# Autodesk Inventor assembly: rcache
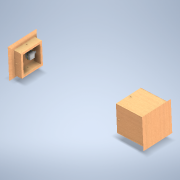
[picture p0: Inventor's stored thumbnail of the model, 180x180]
Saved by Autodesk Inventor 2021 (Build 250183000, 183)
## iProperties
Created: 2020-06-13
Part Number: rcache
Document SubType Name: Assembly
Designer: Yatekii
Author: Yatekii
## Documents named in this file (5)
- C:\Users\Yatekii\repos\rcache\cad\rcache.iam
- C:\Users\Yatekii\repos\rcache\cad\inner.iam
- C:\Users\Yatekii\repos\rcache\cad\outer.iam
- C:\Users\Yatekii\repos\rcache\cad\solenoid\solenoid.iam
- C:\Users\Yatekii\repos\rcache\cad\locker.ipt
## Components (4 placed, 4 different names)
1. inner:1 [sub-assembly] — Slider:1
2. outer:1 [sub-assembly] — Mate:2, Slider:1, Mate:3, Mate:4
3. solenoid:1 [sub-assembly] — Rigid:1, Mate:3, Mate:4
4. locker:1 — Rigid:1, Mate:2
## Relationships (5: Mate 3, WeldJoint 1, TranslationJoint 1)
- Rigid:1 [WeldJoint]: solenoid:1 ↔ locker:1
- Mate:2 (0.5 mm): outer:1 ↔ locker:1
- Slider:1 [TranslationJoint]: inner:1 ↔ outer:1
- Mate:3 (14 mm): outer:1 ↔ solenoid:1
- Mate:4: outer:1 ↔ solenoid:1
